# Autodesk Inventor assembly: Universal Shaft
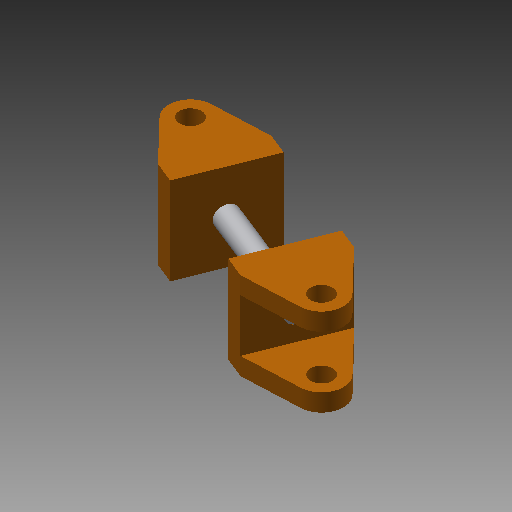
[picture p0: Inventor's stored thumbnail of the model, 512x512]
Saved by Autodesk Inventor 2017 (Build 210142000, 142)
## iProperties
Created: 2014-03-11
Part Number: Universal Shaft
Document SubType Name: Assembly
Designer: John
Author: John
## Documents named in this file (3)
- C:\Users\John Helfen\Desktop\Ex_Files_Invent_2016_EssT\Ex_Files_Invent_2016_EssT\Exercise Files\14_Using constraints to position parts\14_01\Universal Shaft.iam
- C:\Users\John Helfen\Desktop\Ex_Files_Invent_2016_EssT\Ex_Files_Invent_2016_EssT\Exercise Files\14_Using constraints to position parts\14_01\Joint.ipt
- C:\Users\John Helfen\Desktop\Ex_Files_Invent_2016_EssT\Ex_Files_Invent_2016_EssT\Exercise Files\14_Using constraints to position parts\14_01\Connecting Rod.ipt
## Components (3 placed, 2 different names)
1. Joint:1 — Flush:3
2. Joint:2
3. Connecting Rod:1 — Flush:3
## Relationships (5: Flush 3, Mate 2)
- [Mate]: Joint:1 ↔ Joint:2
- [Flush]: Joint:1 ↔ Joint:2
- [Mate]: Joint:1 ↔ Connecting Rod:1
- [Flush]: Joint:2 ↔ Connecting Rod:1
- Flush:3: Joint:1 ↔ Connecting Rod:1
